# Autodesk Inventor assembly: SystemAssemV2
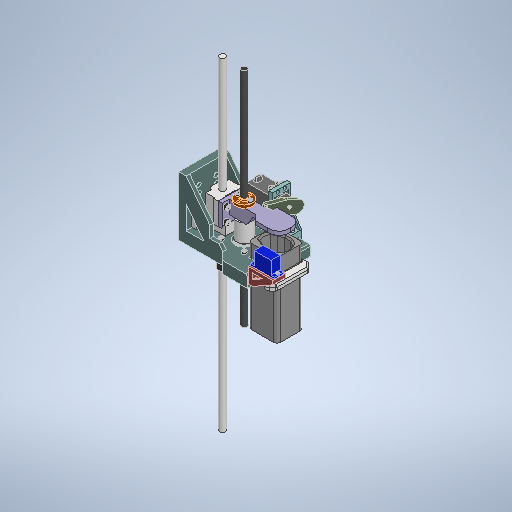
[picture p0: Inventor's stored thumbnail of the model, 512x512]
Saved by Autodesk Inventor 2025.1 (Build 291241000, 241)
## iProperties
Created: 2025-03-02
Part Number: SystemAssemV2
Document SubType Name: Assembly
Designer: 13156
Author: 13156
## Documents named in this file (22)
- C:\Users\13156\OneDrive - Binghamton University\Documents\GitHub\Perovskite-Automated-Synthesis-System\CAD\Pipette\SystemAssemV2.iam
- C:\Users\13156\OneDrive - Binghamton University\Documents\GitHub\Perovskite-Automated-Synthesis-System\CAD\Pipette\HolderV2.ipt
- C:\Users\13156\OneDrive - Binghamton University\Documents\GitHub\Perovskite-Automated-Synthesis-System\CAD\Non 3D Printed Parts\Motors and Servos\NEMA17 Stepper Motor - 26 mm.ipt
- C:\Users\13156\OneDrive - Binghamton University\Documents\GitHub\Perovskite-Automated-Synthesis-System\CAD\Pipette\Pipette Sleeve.ipt
- C:\Users\13156\OneDrive - Binghamton University\Documents\GitHub\Perovskite-Automated-Synthesis-System\CAD\Pipette\LeadScrewBase.ipt
- C:\Users\13156\OneDrive - Binghamton University\Documents\GitHub\Perovskite-Automated-Synthesis-System\CAD\Non 3D Printed Parts\Linear Rails\8mm Linear Rod.ipt
- C:\Users\13156\OneDrive - Binghamton University\Documents\GitHub\Perovskite-Automated-Synthesis-System\CAD\Non 3D Printed Parts\Linear Rails\Linear Bearing 8mm Square.ipt
- C:\Users\13156\OneDrive - Binghamton University\Documents\GitHub\Perovskite-Automated-Synthesis-System\CAD\Pipette\ActuatorV2.ipt
- C:\Users\13156\OneDrive - Binghamton University\Documents\GitHub\Perovskite-Automated-Synthesis-System\CAD\Pipette\BIGServoHolder.ipt
- C:\Users\13156\OneDrive - Binghamton University\Documents\GitHub\Perovskite-Automated-Synthesis-System\CAD\Pipette\996R.ipt
- C:\Users\13156\OneDrive - Binghamton University\Documents\GitHub\Perovskite-Automated-Synthesis-System\CAD\Non 3D Printed Parts\Leadscrew.ipt
- C:\Users\13156\OneDrive - Binghamton University\Documents\GitHub\Perovskite-Automated-Synthesis-System\CAD\Pipette\BigServoEjectorArm.ipt
- C:\Users\13156\OneDrive - Binghamton University\Documents\GitHub\Perovskite-Automated-Synthesis-System\CAD\Non 3D Printed Parts\Threaded Rod 300mm.ipt
- C:\Users\13156\OneDrive - Binghamton University\Documents\GitHub\Perovskite-Automated-Synthesis-System\CAD\Pipette\GrabberServoHolder.ipt
- C:\Users\13156\OneDrive - Binghamton University\Documents\GitHub\Perovskite-Automated-Synthesis-System\CAD\Non 3D Printed Parts\Motors and Servos\SG90 Servo.ipt
- C:\Users\13156\OneDrive - Binghamton University\Documents\GitHub\Perovskite-Automated-Synthesis-System\CAD\Pipette\GrabberArmV2.ipt
- C:\Users\13156\OneDrive - Binghamton University\Documents\GitHub\Perovskite-Automated-Synthesis-System\CAD\Pipette\HalfServoArm.ipt
- C:\Users\13156\OneDrive - Binghamton University\Documents\GitHub\Perovskite-Automated-Synthesis-System\CAD\Non 3D Printed Parts\Linear Rails\Linear Rod Holder SK8.ipt
- C:\Users\13156\OneDrive - Binghamton University\Documents\GitHub\Perovskite-Automated-Synthesis-System\CAD\Non 3D Printed Parts\Screws\M4x20.ipt
- C:\Users\13156\OneDrive - Binghamton University\Documents\GitHub\Perovskite-Automated-Synthesis-System\CAD\Non 3D Printed Parts\Screws\M2x8.ipt
- C:\Users\13156\OneDrive - Binghamton University\Documents\GitHub\Perovskite-Automated-Synthesis-System\CAD\Non 3D Printed Parts\Screws\M3x6.ipt
- C:\Users\13156\OneDrive - Binghamton University\Documents\GitHub\Perovskite-Automated-Synthesis-System\CAD\Non 3D Printed Parts\Screws\M3x8.ipt
## Components (39 placed, 21 different names)
1. HolderV2:1 — Mate:1, Mate:2, Mate:3, Mate:4, Mate:5, Mate:6, Mate:7, Mate:8, Mate:9, Mate:10, Mate:13, Mate:19, Mate:20, Mate:21, Mate:26, Mate:27, Mate:28, Flush:1, Flush:3, Mate:42, Mate:43, Mate:44, Mate:52, Mate:53, Mate:54, Mate:93, Mate:94, Mate:95, Mate:96, Mate:97, Mate:98, Mate:99, Mate:100
2. NEMA17 Stepper Motor - 26 mm:1 — Mate:4, Mate:5, Mate:6, Mate:7, Mate:11, Mate:41
3. Pipette Sleeve:1 — Mate:8, Mate:9, Mate:10
4. LeadScrewBase:1 — Mate:11, Mate:28, Mate:30, Mate:40
5. 8mm Linear Rod:1 — Mate:13, Mate:14, Flush:1
6. Linear Bearing 8mm Square:1 — Mate:14, Mate:16, Mate:29
7. ActuatorV2:1 — Mate:16, Mate:29, Mate:30, Mate:31, Mate:32, Mate:33, Mate:34, Mate:55, Mate:56, Mate:57, Mate:58, Mate:60, Mate:61, Mate:62, Mate:63
8. BIGServoHolder:1 — Mate:19, Mate:20, Mate:21, Mate:24, Mate:26, Mate:27, Mate:36, Mate:37, Mate:72, Mate:73, Mate:74, Mate:75
9. 996R:1 — Mate:24, Mate:36, Mate:37, Mate:38, Mate:39, Mate:84, Mate:85, Mate:86, Mate:87, Mate:88, Mate:89, Mate:90, Mate:91, Mate:92
10. Leadscrew:1 — Mate:31, Mate:32, Mate:33, Mate:34, Mate:40, Mate:80, Mate:81, Mate:82, Mate:83
11. BigServoEjectorArm:1 — Mate:38, Mate:39, Mate:64, Mate:65
12. Threaded Rod 300mm:1 — Mate:41, Flush:3
13. GrabberServoHolder:1 — Mate:42, Mate:43, Mate:44, Mate:45, Mate:46, Mate:47, Mate:68, Mate:69, Mate:70, Mate:71
14. SG90 Servo:1 — Mate:45, Mate:46, Mate:47, Mate:48, Mate:49, Mate:76, Mate:77, Mate:78, Mate:79
15. GrabberArmV2:1 — Mate:50, Mate:51, Mate:59, Mate:66, Mate:67
16. HalfServoArm:1 — Mate:48, Mate:49, Mate:50, Mate:51, Mate:59
17. Linear Rod Holder SK8:1 — Mate:52, Mate:53, Mate:54
18. M4x20:1 — Mate:60, Mate:61
19. M4x20:2 — Mate:62, Mate:63
20. M4x20:3 — Mate:55, Mate:56
21. M4x20:4 — Mate:57, Mate:58
22. M2x8:4 — Mate:66, Mate:67
23. M2x8:5 — Mate:64, Mate:65
24. M2x8:6 — Mate:72, Mate:75
25. M2x8:7 — Mate:73, Mate:74
26. M2x8:8 — Mate:70, Mate:71
27. M2x8:9 — Mate:68, Mate:69
28. M2x8:11 — Mate:76, Mate:79
29. M2x8:12 — Mate:77, Mate:78
30. M3x6:1 — Mate:80, Mate:82
31. M3x6:2 — Mate:81, Mate:83
32. M3x6:3 — Mate:84, Mate:92
33. M3x6:4 — Mate:85, Mate:91
34. M3x6:5 — Mate:87, Mate:88, Mate:90
35. M3x6:6 — Mate:86, Mate:89
36. M3x8:1 — Mate:95, Mate:99
37. M3x8:2 — Mate:94, Mate:97
38. M3x8:3 — Mate:93, Mate:100
39. M3x8:4 — Mate:96, Mate:98
## Relationships (94: Mate 92, Flush 2)
- Mate:1: HolderV2:1
- Mate:2: HolderV2:1
- Mate:3: HolderV2:1
- Mate:4: HolderV2:1 ↔ NEMA17 Stepper Motor - 26 mm:1
- Mate:5: HolderV2:1 ↔ NEMA17 Stepper Motor - 26 mm:1
- Mate:6: HolderV2:1 ↔ NEMA17 Stepper Motor - 26 mm:1
- Mate:7: HolderV2:1 ↔ NEMA17 Stepper Motor - 26 mm:1
- Mate:8: HolderV2:1 ↔ Pipette Sleeve:1
- Mate:9: HolderV2:1 ↔ Pipette Sleeve:1
- Mate:10: HolderV2:1 ↔ Pipette Sleeve:1
- Mate:11: NEMA17 Stepper Motor - 26 mm:1 ↔ LeadScrewBase:1
- Mate:13: HolderV2:1 ↔ 8mm Linear Rod:1
- Mate:14: 8mm Linear Rod:1 ↔ Linear Bearing 8mm Square:1
- Mate:16: Linear Bearing 8mm Square:1 ↔ ActuatorV2:1
- Mate:19: HolderV2:1 ↔ BIGServoHolder:1
- Mate:20: HolderV2:1 ↔ BIGServoHolder:1
- Mate:21: HolderV2:1 ↔ BIGServoHolder:1
- Mate:24: BIGServoHolder:1 ↔ 996R:1
- Mate:26: HolderV2:1 ↔ BIGServoHolder:1
- Mate:27: HolderV2:1 ↔ BIGServoHolder:1
- Mate:28 (2 mm): HolderV2:1 ↔ LeadScrewBase:1
- Flush:1 (-200 mm): HolderV2:1 ↔ 8mm Linear Rod:1
- Mate:29: Linear Bearing 8mm Square:1 ↔ ActuatorV2:1
- Mate:30: LeadScrewBase:1 ↔ ActuatorV2:1
- Mate:31: ActuatorV2:1 ↔ Leadscrew:1
- Mate:32: ActuatorV2:1 ↔ Leadscrew:1
- Mate:33: ActuatorV2:1 ↔ Leadscrew:1
- Mate:34: ActuatorV2:1 ↔ Leadscrew:1
- Mate:36: BIGServoHolder:1 ↔ 996R:1
- Mate:37 (0.5 mm): BIGServoHolder:1 ↔ 996R:1
- Mate:38: 996R:1 ↔ BigServoEjectorArm:1
- Mate:39: 996R:1 ↔ BigServoEjectorArm:1
- Mate:40: LeadScrewBase:1 ↔ Leadscrew:1
- Mate:41: NEMA17 Stepper Motor - 26 mm:1 ↔ Threaded Rod 300mm:1
- Flush:3 (-200 mm): HolderV2:1 ↔ Threaded Rod 300mm:1
- Mate:42: HolderV2:1 ↔ GrabberServoHolder:1
- Mate:43: HolderV2:1 ↔ GrabberServoHolder:1
- Mate:44: HolderV2:1 ↔ GrabberServoHolder:1
- Mate:45: GrabberServoHolder:1 ↔ SG90 Servo:1
- Mate:46: GrabberServoHolder:1 ↔ SG90 Servo:1
- Mate:47: GrabberServoHolder:1 ↔ SG90 Servo:1
- Mate:48: SG90 Servo:1 ↔ HalfServoArm:1
- Mate:49 (1 mm): SG90 Servo:1 ↔ HalfServoArm:1
- Mate:50: GrabberArmV2:1 ↔ HalfServoArm:1
- Mate:51: GrabberArmV2:1 ↔ HalfServoArm:1
- Mate:52: HolderV2:1 ↔ Linear Rod Holder SK8:1
- Mate:53: HolderV2:1 ↔ Linear Rod Holder SK8:1
- Mate:54: HolderV2:1 ↔ Linear Rod Holder SK8:1
- Mate:55: ActuatorV2:1 ↔ M4x20:3
- Mate:56: ActuatorV2:1 ↔ M4x20:3
- Mate:57: ActuatorV2:1 ↔ M4x20:4
- Mate:58: ActuatorV2:1 ↔ M4x20:4
- Mate:59: GrabberArmV2:1 ↔ HalfServoArm:1
- Mate:60: ActuatorV2:1 ↔ M4x20:1
- Mate:61: ActuatorV2:1 ↔ M4x20:1
- Mate:62: ActuatorV2:1 ↔ M4x20:2
- Mate:63: ActuatorV2:1 ↔ M4x20:2
- Mate:64: BigServoEjectorArm:1 ↔ M2x8:5
- Mate:65: BigServoEjectorArm:1 ↔ M2x8:5
- Mate:66: GrabberArmV2:1 ↔ M2x8:4
- Mate:67: GrabberArmV2:1 ↔ M2x8:4
- Mate:68: GrabberServoHolder:1 ↔ M2x8:9
- Mate:69: GrabberServoHolder:1 ↔ M2x8:9
- Mate:70: GrabberServoHolder:1 ↔ M2x8:8
- Mate:71: GrabberServoHolder:1 ↔ M2x8:8
- Mate:72: BIGServoHolder:1 ↔ M2x8:6
- Mate:73: BIGServoHolder:1 ↔ M2x8:7
- Mate:74: BIGServoHolder:1 ↔ M2x8:7
- Mate:75: BIGServoHolder:1 ↔ M2x8:6
- Mate:76: SG90 Servo:1 ↔ M2x8:11
- Mate:77: SG90 Servo:1 ↔ M2x8:12
- Mate:78: SG90 Servo:1 ↔ M2x8:12
- Mate:79: SG90 Servo:1 ↔ M2x8:11
- Mate:80: Leadscrew:1 ↔ M3x6:1
- Mate:81: Leadscrew:1 ↔ M3x6:2
- Mate:82: Leadscrew:1 ↔ M3x6:1
- Mate:83: Leadscrew:1 ↔ M3x6:2
- Mate:84: 996R:1 ↔ M3x6:3
- Mate:85: 996R:1 ↔ M3x6:4
- Mate:86: 996R:1 ↔ M3x6:6
- Mate:87: 996R:1 ↔ M3x6:5
- Mate:88: 996R:1 ↔ M3x6:5
- Mate:89: 996R:1 ↔ M3x6:6
- Mate:90: 996R:1 ↔ M3x6:5
- Mate:91: 996R:1 ↔ M3x6:4
- Mate:92: 996R:1 ↔ M3x6:3
- Mate:93: HolderV2:1 ↔ M3x8:3
- Mate:94: HolderV2:1 ↔ M3x8:2
- Mate:95: HolderV2:1 ↔ M3x8:1
- Mate:96: HolderV2:1 ↔ M3x8:4
- Mate:97: HolderV2:1 ↔ M3x8:2
- Mate:98: HolderV2:1 ↔ M3x8:4
- Mate:99: HolderV2:1 ↔ M3x8:1
- Mate:100: HolderV2:1 ↔ M3x8:3
